# Autodesk Inventor assembly: Bionic_Hand_Baugruppe_Version_1
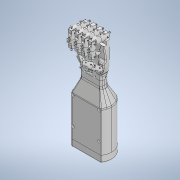
[picture p0: Inventor's stored thumbnail of the model, 180x180]
Saved by Autodesk Inventor 2021 (Build 250183000, 183)
## iProperties
Created: 2021-05-12
Part Number: Bionic_Hand_Baugruppe_Version_1
Document SubType Name: Assembly
Designer: Maxim
Author: Maxim
## Documents named in this file (18)
- D:\MEDS Studium\4. Semester\Informatik IV\Bionic Hand Version 1.1\Bionic_Hand_Baugruppe_Version_1.iam
- D:\MEDS Studium\4. Semester\Informatik IV\Bionic Hand Version 1.1\Handkörper.ipt
- D:\MEDS Studium\4. Semester\Informatik IV\Bionic Hand Version 1.1\Finger_Baugruppe.iam
- D:\MEDS Studium\4. Semester\Informatik IV\Bionic Hand Version 1.1\Daumen_Baugruppe.iam
- D:\MEDS Studium\4. Semester\Informatik IV\Bionic Hand Version 1.1\din_en_iso_4762_m3x10.ipt
- D:\MEDS Studium\4. Semester\Informatik IV\Bionic Hand Version 1.1\Unterarm_Teil_1.ipt
- D:\MEDS Studium\4. Semester\Informatik IV\Bionic Hand Version 1.1\SG90 - Micro Servo 9g - Tower Pro.1.ipt
- D:\MEDS Studium\4. Semester\Informatik IV\Bionic Hand Version 1.1\Servo_Rad_20_Durchmesser.ipt
- D:\MEDS Studium\4. Semester\Informatik IV\Bionic Hand Version 1.1\Unterarm_Teil_2.ipt
- D:\MEDS Studium\4. Semester\Informatik IV\Bionic Hand Version 1.1\Unterarm_Verschluss.ipt
- D:\MEDS Studium\4. Semester\Informatik IV\Bionic Hand Version 1.1\Lochrasterplatine.ipt
- D:\MEDS Studium\4. Semester\Informatik IV\Bionic Hand Version 1.1\din_en_iso_4762_m2x4.ipt
- D:\MEDS Studium\4. Semester\Informatik IV\Bionic Hand Version 1.1\din_en_iso_4762_m5x12.ipt
- D:\MEDS Studium\4. Semester\Informatik IV\Bionic Hand Version 1.1\din_en_iso_4762_m3x12.ipt
- D:\MEDS Studium\4. Semester\Informatik IV\Bionic Hand Version 1.1\din_en_iso_4762_m3x8.ipt
- D:\MEDS Studium\4. Semester\Informatik IV\Bionic Hand Version 1.1\din_en_iso_4762_m5x40.ipt
- D:\MEDS Studium\4. Semester\Informatik IV\Bionic Hand Version 1.1\din_en_iso_4762_m5x30.ipt
- D:\MEDS Studium\4. Semester\Informatik IV\Bionic Hand Version 1.1\Faden_Halter_24_Durchmesser.ipt
## Components (61 placed, 17 different names)
1. Handkörper:1 — Passend:11, Passend:12, Passend:13, Passend:14, Passend:16, Passend:17, Passend:18, Passend:19, Passend:20, Passend:21, Passend:22, Passend:46, Passend:48, Passend:49, Passend:50, Passend:72, Fluchtend:48, Passend:81, Passend:82, Passend:83, Passend:84, Passend:85, Passend:86, Passend:87, Passend:88, Passend:89, Passend:90, Passend:91, Passend:92, Passend:93, Passend:94, Passend:95, Passend:96, Passend:97, Passend:98, Passend:99, Passend:100, Passend:101, Passend:102, Passend:103, Passend:104, Passend:105, Passend:106, Zylindrisch:16, Zylindrisch:12, Zylindrisch:13, Zylindrisch:14, Passend:123, Passend:124, Passend:125, Zylindrisch:15
2. Finger_Baugruppe:1 [sub-assembly] — Passend:50, Zylindrisch:14
3. Finger_Baugruppe:2 [sub-assembly] — Passend:49, Zylindrisch:13
4. Finger_Baugruppe:3 [sub-assembly] — Passend:48, Zylindrisch:12
5. Finger_Baugruppe:4 [sub-assembly] — Passend:46, Zylindrisch:16
6. Daumen_Baugruppe:1 [sub-assembly] — Passend:123, Zylindrisch:15
7. din_en_iso_4762_m3x10:1 — Passend:14, Passend:19
8. din_en_iso_4762_m3x10:2 — Passend:13, Passend:18
9. din_en_iso_4762_m3x10:3 — Passend:12, Passend:17
10. din_en_iso_4762_m3x10:4 — Passend:11, Passend:16
11. din_en_iso_4762_m3x10:5 — Passend:124, Passend:125
12. SG90 - Micro Servo 9g - Tower Pro.1:1 — Passend:55, Passend:56, Passend:144, Passend:145, Passend:146
13. SG90 - Micro Servo 9g - Tower Pro.1:2 — Passend:53, Passend:54, Passend:126, Passend:147, Passend:148, Passend:149
14. SG90 - Micro Servo 9g - Tower Pro.1:3 — Passend:34, Passend:35, Passend:36, Passend:141, Passend:156, Passend:157, Passend:158
15. SG90 - Micro Servo 9g - Tower Pro.1:4 — Passend:51, Passend:52, Passend:137, Passend:153, Passend:154, Passend:155
16. SG90 - Micro Servo 9g - Tower Pro.1:5 — Passend:57, Passend:58, Passend:130, Passend:150, Passend:151, Passend:152
17. Servo_Rad_20_Durchmesser:2 — Passend:34, Fluchtend:6, Passend:35, Fluchtend:47, Passend:139, Passend:140
18. Servo_Rad_20_Durchmesser:1 — Passend:55, Passend:56, Passend:68, Passend:69, Passend:70, Passend:77, Passend:78
19. Servo_Rad_20_Durchmesser:4 — Passend:53, Passend:54, Passend:62, Passend:63, Passend:64, Passend:127
20. Servo_Rad_20_Durchmesser:3 — Passend:51, Passend:52, Passend:59, Passend:60, Passend:61, Passend:135, Passend:136
21. Servo_Rad_20_Durchmesser:5 — Passend:57, Passend:58, Passend:131, Passend:133, Passend:142, Passend:143, Passend:159
22. Faden_Halter_24_Durchmesser:1 — Passend:59, Passend:60, Passend:61, Passend:134
23. Faden_Halter_24_Durchmesser:2 — Passend:62, Passend:63, Passend:64, Passend:128, Passend:129
24. Faden_Halter_24_Durchmesser:3 — Passend:142, Passend:143, Passend:159, Passend:160
25. Faden_Halter_24_Durchmesser:4 — Fluchtend:6, Passend:36, Fluchtend:47, Passend:138
26. Faden_Halter_24_Durchmesser:5 — Passend:68, Passend:69, Passend:70, Passend:75, Passend:76
27. Unterarm_Teil_1:1 — Passend:20, Passend:21, Passend:22, Passend:71, Passend:74, Passend:144, Passend:145, Passend:146, Passend:147, Passend:148, Passend:149, Passend:150, Passend:151, Passend:152, Passend:153, Passend:154, Passend:155, Passend:156, Passend:157, Passend:158, Fluchtend:50, Passend:161
28. Unterarm_Teil_2:1 — Passend:71, Passend:72, Fluchtend:48, Fluchtend:49, Passend:107, Passend:108, Passend:109, Passend:110, Passend:111, Passend:112, Passend:113, Passend:114
29. Unterarm_Verschluss:1 — Fluchtend:49, Passend:73, Passend:115, Passend:116, Passend:117, Passend:118, Passend:119, Passend:120, Passend:121, Passend:122, Fluchtend:50, Passend:161, Passend:162, Fluchtend:51, Passend:163
30. Lochrasterplatine_60x40:1 — Passend:73, Passend:74
31. din_en_iso_4762_m5x12:1 — Passend:81, Passend:82
32. din_en_iso_4762_m5x12:2 — Passend:83, Passend:84
33. din_en_iso_4762_m5x12:3 — Passend:87, Passend:94
34. din_en_iso_4762_m5x12:4 — Passend:85, Passend:86
35. din_en_iso_4762_m3x12:1 — Passend:92, Passend:93
36. din_en_iso_4762_m3x12:2 — Passend:90, Passend:91
37. din_en_iso_4762_m3x12:3 — Passend:88, Passend:89
38. din_en_iso_4762_m3x8:1 — Passend:95, Passend:96
39. din_en_iso_4762_m3x8:2 — Passend:97, Passend:98
40. din_en_iso_4762_m3x8:3 — Passend:99, Passend:100
41. din_en_iso_4762_m3x8:4 — Passend:101, Passend:102
42. din_en_iso_4762_m3x8:5 — Passend:103, Passend:104
43. din_en_iso_4762_m3x8:6 — Passend:105, Passend:106
44. din_en_iso_4762_m5x40:1 — Passend:107, Passend:108
45. din_en_iso_4762_m5x40:2 — Passend:113, Passend:114
46. din_en_iso_4762_m5x40:3 — Passend:111, Passend:112
47. din_en_iso_4762_m5x40:4 — Passend:109, Passend:110
48. din_en_iso_4762_m5x30:1 — Passend:117, Passend:118
49. din_en_iso_4762_m5x30:2 — Passend:121, Passend:122
50. din_en_iso_4762_m5x30:3 — Passend:119, Passend:120
51. din_en_iso_4762_m5x30:4 — Passend:115, Passend:116
52. din_en_iso_4762_m2x4:1 — Passend:75, Passend:76
53. din_en_iso_4762_m2x4:2 — Passend:77, Passend:78
54. din_en_iso_4762_m2x4:3 — Passend:126, Passend:127
55. din_en_iso_4762_m2x4:4 — Passend:128, Passend:129
56. din_en_iso_4762_m2x4:5 — Passend:130, Passend:131
57. din_en_iso_4762_m2x4:6 — Passend:133, Passend:160
58. din_en_iso_4762_m2x4:7 — Passend:134, Passend:135
59. din_en_iso_4762_m2x4:8 — Passend:136, Passend:137
60. din_en_iso_4762_m2x4:9 — Passend:138, Passend:139
61. din_en_iso_4762_m2x4:10 — Passend:140, Passend:141
## Relationships (136: Mate 125, Flush 6, CylindricalJoint 5)
- Passend:11 [Mate]: Handkörper:1 ↔ din_en_iso_4762_m3x10:4
- Passend:12 [Mate]: Handkörper:1 ↔ din_en_iso_4762_m3x10:3
- Passend:13 [Mate]: Handkörper:1 ↔ din_en_iso_4762_m3x10:2
- Passend:14 [Mate]: Handkörper:1 ↔ din_en_iso_4762_m3x10:1
- Passend:16 [Mate]: Handkörper:1 ↔ din_en_iso_4762_m3x10:4
- Passend:17 [Mate]: Handkörper:1 ↔ din_en_iso_4762_m3x10:3
- Passend:18 [Mate]: Handkörper:1 ↔ din_en_iso_4762_m3x10:2
- Passend:19 [Mate]: Handkörper:1 ↔ din_en_iso_4762_m3x10:1
- Passend:20 [Mate]: Handkörper:1 ↔ Unterarm_Teil_1:1
- Passend:21 [Mate]: Handkörper:1 ↔ Unterarm_Teil_1:1
- Passend:22 [Mate]: Handkörper:1 ↔ Unterarm_Teil_1:1
- Passend:34 [Mate]: SG90 - Micro Servo 9g - Tower Pro.1:3 ↔ Servo_Rad_20_Durchmesser:2
- Fluchtend:6 [Flush]: Servo_Rad_20_Durchmesser:2 ↔ Faden_Halter_24_Durchmesser:4
- Passend:35 [Mate]: SG90 - Micro Servo 9g - Tower Pro.1:3 ↔ Servo_Rad_20_Durchmesser:2
- Passend:36 [Mate]: SG90 - Micro Servo 9g - Tower Pro.1:3 ↔ Faden_Halter_24_Durchmesser:4
- Fluchtend:47 [Flush]: Servo_Rad_20_Durchmesser:2 ↔ Faden_Halter_24_Durchmesser:4
- Passend:46 [Mate] (0.2 mm): Handkörper:1 ↔ Finger_Baugruppe:4
- Passend:48 [Mate] (0.2 mm): Handkörper:1 ↔ Finger_Baugruppe:3
- Passend:49 [Mate] (0.2 mm): Handkörper:1 ↔ Finger_Baugruppe:2
- Passend:50 [Mate] (0.2 mm): Handkörper:1 ↔ Finger_Baugruppe:1
- Passend:51 [Mate]: SG90 - Micro Servo 9g - Tower Pro.1:4 ↔ Servo_Rad_20_Durchmesser:3
- Passend:52 [Mate]: SG90 - Micro Servo 9g - Tower Pro.1:4 ↔ Servo_Rad_20_Durchmesser:3
- Passend:53 [Mate]: SG90 - Micro Servo 9g - Tower Pro.1:2 ↔ Servo_Rad_20_Durchmesser:4
- Passend:54 [Mate]: SG90 - Micro Servo 9g - Tower Pro.1:2 ↔ Servo_Rad_20_Durchmesser:4
- Passend:55 [Mate]: SG90 - Micro Servo 9g - Tower Pro.1:1 ↔ Servo_Rad_20_Durchmesser:1
- Passend:56 [Mate]: SG90 - Micro Servo 9g - Tower Pro.1:1 ↔ Servo_Rad_20_Durchmesser:1
- Passend:57 [Mate]: SG90 - Micro Servo 9g - Tower Pro.1:5 ↔ Servo_Rad_20_Durchmesser:5
- Passend:58 [Mate]: SG90 - Micro Servo 9g - Tower Pro.1:5 ↔ Servo_Rad_20_Durchmesser:5
- Passend:59 [Mate]: Servo_Rad_20_Durchmesser:3 ↔ Faden_Halter_24_Durchmesser:1
- Passend:60 [Mate]: Servo_Rad_20_Durchmesser:3 ↔ Faden_Halter_24_Durchmesser:1
- Passend:61 [Mate]: Servo_Rad_20_Durchmesser:3 ↔ Faden_Halter_24_Durchmesser:1
- Passend:62 [Mate]: Servo_Rad_20_Durchmesser:4 ↔ Faden_Halter_24_Durchmesser:2
- Passend:63 [Mate]: Servo_Rad_20_Durchmesser:4 ↔ Faden_Halter_24_Durchmesser:2
- Passend:64 [Mate]: Servo_Rad_20_Durchmesser:4 ↔ Faden_Halter_24_Durchmesser:2
- Passend:68 [Mate]: Servo_Rad_20_Durchmesser:1 ↔ Faden_Halter_24_Durchmesser:5
- Passend:69 [Mate]: Servo_Rad_20_Durchmesser:1 ↔ Faden_Halter_24_Durchmesser:5
- Passend:70 [Mate]: Servo_Rad_20_Durchmesser:1 ↔ Faden_Halter_24_Durchmesser:5
- Passend:71 [Mate]: Unterarm_Teil_1:1 ↔ Unterarm_Teil_2:1
- Passend:72 [Mate]: Handkörper:1 ↔ Unterarm_Teil_2:1
- Fluchtend:48 [Flush]: Handkörper:1 ↔ Unterarm_Teil_2:1
- Fluchtend:49 [Flush]: Unterarm_Teil_2:1 ↔ Unterarm_Verschluss:1
- Passend:73 [Mate] (3 mm): Unterarm_Verschluss:1 ↔ Lochrasterplatine_60x40:1
- Passend:74 [Mate] (4.5 mm): Unterarm_Teil_1:1 ↔ Lochrasterplatine_60x40:1
- Passend:75 [Mate]: Faden_Halter_24_Durchmesser:5 ↔ din_en_iso_4762_m2x4:1
- Passend:76 [Mate]: Faden_Halter_24_Durchmesser:5 ↔ din_en_iso_4762_m2x4:1
- Passend:77 [Mate]: Servo_Rad_20_Durchmesser:1 ↔ din_en_iso_4762_m2x4:2
- Passend:78 [Mate]: Servo_Rad_20_Durchmesser:1 ↔ din_en_iso_4762_m2x4:2
- Passend:81 [Mate]: Handkörper:1 ↔ din_en_iso_4762_m5x12:1
- Passend:82 [Mate]: Handkörper:1 ↔ din_en_iso_4762_m5x12:1
- Passend:83 [Mate]: Handkörper:1 ↔ din_en_iso_4762_m5x12:2
- Passend:84 [Mate]: Handkörper:1 ↔ din_en_iso_4762_m5x12:2
- Passend:85 [Mate]: Handkörper:1 ↔ din_en_iso_4762_m5x12:4
- Passend:86 [Mate]: Handkörper:1 ↔ din_en_iso_4762_m5x12:4
- Passend:87 [Mate]: Handkörper:1 ↔ din_en_iso_4762_m5x12:3
- Passend:88 [Mate]: Handkörper:1 ↔ din_en_iso_4762_m3x12:3
- Passend:89 [Mate]: Handkörper:1 ↔ din_en_iso_4762_m3x12:3
- Passend:90 [Mate]: Handkörper:1 ↔ din_en_iso_4762_m3x12:2
- Passend:91 [Mate]: Handkörper:1 ↔ din_en_iso_4762_m3x12:2
- Passend:92 [Mate]: Handkörper:1 ↔ din_en_iso_4762_m3x12:1
- Passend:93 [Mate]: Handkörper:1 ↔ din_en_iso_4762_m3x12:1
- Passend:94 [Mate]: Handkörper:1 ↔ din_en_iso_4762_m5x12:3
- Passend:95 [Mate]: Handkörper:1 ↔ din_en_iso_4762_m3x8:1
- Passend:96 [Mate]: Handkörper:1 ↔ din_en_iso_4762_m3x8:1
- Passend:97 [Mate]: Handkörper:1 ↔ din_en_iso_4762_m3x8:2
- Passend:98 [Mate]: Handkörper:1 ↔ din_en_iso_4762_m3x8:2
- Passend:99 [Mate]: Handkörper:1 ↔ din_en_iso_4762_m3x8:3
- Passend:100 [Mate]: Handkörper:1 ↔ din_en_iso_4762_m3x8:3
- Passend:101 [Mate]: Handkörper:1 ↔ din_en_iso_4762_m3x8:4
- Passend:102 [Mate]: Handkörper:1 ↔ din_en_iso_4762_m3x8:4
- Passend:103 [Mate]: Handkörper:1 ↔ din_en_iso_4762_m3x8:5
- Passend:104 [Mate]: Handkörper:1 ↔ din_en_iso_4762_m3x8:5
- Passend:105 [Mate]: Handkörper:1 ↔ din_en_iso_4762_m3x8:6
- Passend:106 [Mate]: Handkörper:1 ↔ din_en_iso_4762_m3x8:6
- Passend:107 [Mate]: Unterarm_Teil_2:1 ↔ din_en_iso_4762_m5x40:1
- Passend:108 [Mate]: Unterarm_Teil_2:1 ↔ din_en_iso_4762_m5x40:1
- Passend:109 [Mate]: Unterarm_Teil_2:1 ↔ din_en_iso_4762_m5x40:4
- Passend:110 [Mate]: Unterarm_Teil_2:1 ↔ din_en_iso_4762_m5x40:4
- Passend:111 [Mate]: Unterarm_Teil_2:1 ↔ din_en_iso_4762_m5x40:3
- Passend:112 [Mate]: Unterarm_Teil_2:1 ↔ din_en_iso_4762_m5x40:3
- Passend:113 [Mate]: Unterarm_Teil_2:1 ↔ din_en_iso_4762_m5x40:2
- Passend:114 [Mate]: Unterarm_Teil_2:1 ↔ din_en_iso_4762_m5x40:2
- Passend:115 [Mate]: Unterarm_Verschluss:1 ↔ din_en_iso_4762_m5x30:4
- Passend:116 [Mate]: Unterarm_Verschluss:1 ↔ din_en_iso_4762_m5x30:4
- Passend:117 [Mate]: Unterarm_Verschluss:1 ↔ din_en_iso_4762_m5x30:1
- Passend:118 [Mate]: Unterarm_Verschluss:1 ↔ din_en_iso_4762_m5x30:1
- Passend:119 [Mate]: Unterarm_Verschluss:1 ↔ din_en_iso_4762_m5x30:3
- Passend:120 [Mate]: Unterarm_Verschluss:1 ↔ din_en_iso_4762_m5x30:3
- Passend:121 [Mate]: Unterarm_Verschluss:1 ↔ din_en_iso_4762_m5x30:2
- Passend:122 [Mate]: Unterarm_Verschluss:1 ↔ din_en_iso_4762_m5x30:2
- Zylindrisch:16 [CylindricalJoint]: Handkörper:1 ↔ Finger_Baugruppe:4
- Zylindrisch:12 [CylindricalJoint]: Handkörper:1 ↔ Finger_Baugruppe:3
- Zylindrisch:13 [CylindricalJoint]: Handkörper:1 ↔ Finger_Baugruppe:2
- Zylindrisch:14 [CylindricalJoint]: Handkörper:1 ↔ Finger_Baugruppe:1
- Passend:123 [Mate] (-4.8 mm): Handkörper:1 ↔ Daumen_Baugruppe:1
- Passend:124 [Mate]: Handkörper:1 ↔ din_en_iso_4762_m3x10:5
- Passend:125 [Mate]: Handkörper:1 ↔ din_en_iso_4762_m3x10:5
- Zylindrisch:15 [CylindricalJoint]: Handkörper:1 ↔ Daumen_Baugruppe:1
- Passend:126 [Mate]: SG90 - Micro Servo 9g - Tower Pro.1:2 ↔ din_en_iso_4762_m2x4:3
- Passend:127 [Mate]: Servo_Rad_20_Durchmesser:4 ↔ din_en_iso_4762_m2x4:3
- Passend:128 [Mate]: Faden_Halter_24_Durchmesser:2 ↔ din_en_iso_4762_m2x4:4
- Passend:129 [Mate]: Faden_Halter_24_Durchmesser:2 ↔ din_en_iso_4762_m2x4:4
- Passend:130 [Mate]: SG90 - Micro Servo 9g - Tower Pro.1:5 ↔ din_en_iso_4762_m2x4:5
- Passend:131 [Mate]: Servo_Rad_20_Durchmesser:5 ↔ din_en_iso_4762_m2x4:5
- Passend:133 [Mate]: Servo_Rad_20_Durchmesser:5 ↔ din_en_iso_4762_m2x4:6
- Passend:134 [Mate]: Faden_Halter_24_Durchmesser:1 ↔ din_en_iso_4762_m2x4:7
- Passend:135 [Mate]: Servo_Rad_20_Durchmesser:3 ↔ din_en_iso_4762_m2x4:7
- Passend:136 [Mate]: Servo_Rad_20_Durchmesser:3 ↔ din_en_iso_4762_m2x4:8
- Passend:137 [Mate]: SG90 - Micro Servo 9g - Tower Pro.1:4 ↔ din_en_iso_4762_m2x4:8
- Passend:138 [Mate]: Faden_Halter_24_Durchmesser:4 ↔ din_en_iso_4762_m2x4:9
- Passend:139 [Mate]: Servo_Rad_20_Durchmesser:2 ↔ din_en_iso_4762_m2x4:9
- Passend:140 [Mate]: Servo_Rad_20_Durchmesser:2 ↔ din_en_iso_4762_m2x4:10
- Passend:141 [Mate]: SG90 - Micro Servo 9g - Tower Pro.1:3 ↔ din_en_iso_4762_m2x4:10
- Passend:142 [Mate]: Servo_Rad_20_Durchmesser:5 ↔ Faden_Halter_24_Durchmesser:3
- Passend:143 [Mate]: Servo_Rad_20_Durchmesser:5 ↔ Faden_Halter_24_Durchmesser:3
- Passend:144 [Mate]: SG90 - Micro Servo 9g - Tower Pro.1:1 ↔ Unterarm_Teil_1:1
- Passend:145 [Mate]: SG90 - Micro Servo 9g - Tower Pro.1:1 ↔ Unterarm_Teil_1:1
- Passend:146 [Mate]: SG90 - Micro Servo 9g - Tower Pro.1:1 ↔ Unterarm_Teil_1:1
- Passend:147 [Mate]: SG90 - Micro Servo 9g - Tower Pro.1:2 ↔ Unterarm_Teil_1:1
- Passend:148 [Mate]: SG90 - Micro Servo 9g - Tower Pro.1:2 ↔ Unterarm_Teil_1:1
- Passend:149 [Mate]: SG90 - Micro Servo 9g - Tower Pro.1:2 ↔ Unterarm_Teil_1:1
- Passend:150 [Mate]: SG90 - Micro Servo 9g - Tower Pro.1:5 ↔ Unterarm_Teil_1:1
- Passend:151 [Mate]: SG90 - Micro Servo 9g - Tower Pro.1:5 ↔ Unterarm_Teil_1:1
- Passend:152 [Mate]: SG90 - Micro Servo 9g - Tower Pro.1:5 ↔ Unterarm_Teil_1:1
- Passend:153 [Mate]: SG90 - Micro Servo 9g - Tower Pro.1:4 ↔ Unterarm_Teil_1:1
- Passend:154 [Mate]: SG90 - Micro Servo 9g - Tower Pro.1:4 ↔ Unterarm_Teil_1:1
- Passend:155 [Mate]: SG90 - Micro Servo 9g - Tower Pro.1:4 ↔ Unterarm_Teil_1:1
- Passend:156 [Mate]: SG90 - Micro Servo 9g - Tower Pro.1:3 ↔ Unterarm_Teil_1:1
- Passend:157 [Mate]: SG90 - Micro Servo 9g - Tower Pro.1:3 ↔ Unterarm_Teil_1:1
- Passend:158 [Mate]: SG90 - Micro Servo 9g - Tower Pro.1:3 ↔ Unterarm_Teil_1:1
- Passend:159 [Mate]: Servo_Rad_20_Durchmesser:5 ↔ Faden_Halter_24_Durchmesser:3
- Passend:160 [Mate]: Faden_Halter_24_Durchmesser:3 ↔ din_en_iso_4762_m2x4:6
- Fluchtend:50 [Flush]: Unterarm_Teil_1:1 ↔ Unterarm_Verschluss:1
- Passend:161 [Mate]: Unterarm_Teil_1:1 ↔ Unterarm_Verschluss:1
- Passend:162 [Mate]: Unterarm_Verschluss:1
- Fluchtend:51 [Flush]: Unterarm_Verschluss:1
- Passend:163 [Mate] (-13.5 mm): Unterarm_Verschluss:1
